# Autodesk Inventor assembly: Purple_Reign
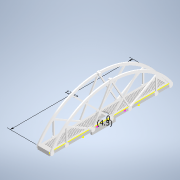
[picture p0: Inventor's stored thumbnail of the model, 180x180]
Saved by Autodesk Inventor 2022.1 (Build 261234000, 234)
## iProperties
Created: 2023-05-01
Part Number: Purple_Reign
Document SubType Name: Assembly
Designer: edgar_tejada0971
Author: edgar_tejada0971
## Documents named in this file (5)
- C:\Users\edgar_tejada0971\Documents\Purple_Reign\Bridge\Purple_Reign.iam
- C:\Users\edgar_tejada0971\Documents\Purple_Reign\Bridge\purple reign bridge.ipt
- C:\Users\edgar_tejada0971\Documents\Purple_Reign\Bridge\East_Side.ipt
- C:\Users\edgar_tejada0971\Documents\Purple_Reign\Bridge\purple reign bridge_MIR.ipt
- C:\Users\edgar_tejada0971\Documents\Purple_Reign\Bridge\West_Side.ipt
## Components (6 placed, 4 different names)
1. purple reign bridge:1 — Insert:1, Insert:3, Flush:1, Insert:4
2. East_Side:1 — Insert:1
3. purple reign bridge_MIR:1 — Insert:2, Insert:3, Flush:1, Insert:5
4. West_Side:1 — Insert:2
5. West_Side:2 — Insert:4
6. East_Side:2 — Insert:5
## Relationships (6: Insert 5, Flush 1)
- Insert:1: purple reign bridge:1 ↔ East_Side:1
- Insert:2: purple reign bridge_MIR:1 ↔ West_Side:1
- Insert:3: purple reign bridge:1 ↔ purple reign bridge_MIR:1
- Flush:1: purple reign bridge:1 ↔ purple reign bridge_MIR:1
- Insert:4: purple reign bridge:1 ↔ West_Side:2
- Insert:5 (-4 mm): purple reign bridge_MIR:1 ↔ East_Side:2
